# Autodesk Inventor assembly: CapForWater
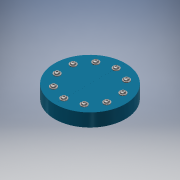
[picture p0: Inventor's stored thumbnail of the model, 180x180]
Saved by Autodesk Inventor 2019 (Build 230136000, 136)
## iProperties
Created: 2017-11-20
Part Number: CapForWater
Document SubType Name: Assembly
Designer: steele
Author: steele
## Documents named in this file (4)
- C:\git\CAD-Development\robSteele\HouseProjects\Garage\CapForWater.iam
- C:\git\CAD-Development\robSteele\HouseProjects\Garage\CoverPlateForWaterHalf.ipt
- C:\git\CAD-Development\robSteele\HouseProjects\Garage\SupportPlateForWater.ipt
- C:\git\CAD-Development\robSteele\HouseProjects\Garage\CapForWater\Design Accelerator\Bolted Connection3.iam
## Components (4 placed, 3 different names)
1. CoverPlateForWaterHalf:1 — Mate:1, Mate:2, Mate:3, Insert:2, Mate:4, Mate:5
2. CoverPlateForWaterHalf:2 — Mate:1, Mate:2, Mate:3, Insert:1
3. SupportPlateForWater:1 — Insert:1, Insert:2
4. Bolted Connection:1 [sub-assembly] — Mate:4, Mate:5
## Relationships (7: Mate 5, Insert 2)
- Mate:1: CoverPlateForWaterHalf:1 ↔ CoverPlateForWaterHalf:2
- Mate:2: CoverPlateForWaterHalf:1 ↔ CoverPlateForWaterHalf:2
- Mate:3: CoverPlateForWaterHalf:1 ↔ CoverPlateForWaterHalf:2
- Insert:1: CoverPlateForWaterHalf:2 ↔ SupportPlateForWater:1
- Insert:2: CoverPlateForWaterHalf:1 ↔ SupportPlateForWater:1
- Mate:4: CoverPlateForWaterHalf:1 ↔ Bolted Connection:1
- Mate:5: CoverPlateForWaterHalf:1 ↔ Bolted Connection:1
